# Autodesk Inventor assembly: Assembly1
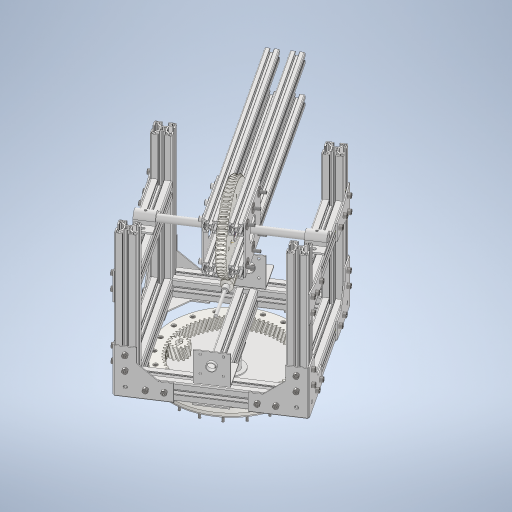
[picture p0: Inventor's stored thumbnail of the model, 512x512]
Saved by Autodesk Inventor 2024 (Build 280153000, 153)
## iProperties
Created: 2025-12-08
Part Number: Assembly1
Document SubType Name: Assembly
Designer: schar
Author: schar
## Documents named in this file (30)
- C:\Users\schar\Desktop\projectBlueprint\AMSTS\hardware\Assembly1.iam
- C:\Users\schar\Desktop\projectBlueprint\AMSTS\hardware\3030_200.ipt
- C:\Users\schar\Desktop\projectBlueprint\AMSTS\hardware\Connect2x3030_m6.ipt
- C:\Users\schar\Desktop\projectBlueprint\AMSTS\hardware\3030_tnut_m6.ipt
- C:\Users\schar\Documents\Inventor\Content Center Files\R2024\en-US\AS 1420\AS 1420 - 1973 - M5 x 10.ipt
- C:\Users\schar\Desktop\projectBlueprint\AMSTS\hardware\3030_260.ipt
- C:\Users\schar\Desktop\projectBlueprint\AMSTS\hardware\3030_connector_assembled.iam
- C:\Users\schar\Desktop\projectBlueprint\AMSTS\hardware\3030_connector_assembled_MIR.iam
- C:\Users\schar\Desktop\projectBlueprint\AMSTS\hardware\3030_connector_assembled_MIR1.iam
- C:\Users\schar\Desktop\projectBlueprint\AMSTS\hardware\3030_connector_assembled_MIR_MIR.iam
- C:\Users\schar\Desktop\projectBlueprint\AMSTS\hardware\3030_T_connector_assembled.iam
- C:\Users\schar\Desktop\projectBlueprint\AMSTS\hardware\3030_T_connector_assembled_MIR1.iam
- C:\Users\schar\Desktop\projectBlueprint\AMSTS\hardware\NEMA 17 - MS17HD2.iam
- C:\Users\schar\Desktop\projectBlueprint\AMSTS\hardware\wormgear_pol_base.iam
- C:\Users\schar\Desktop\projectBlueprint\AMSTS\hardware\base_axis_static_12mm.ipt
- C:\Users\schar\Desktop\projectBlueprint\AMSTS\hardware\base_axis_12mm.ipt
- C:\Users\schar\Desktop\projectBlueprint\AMSTS\hardware\NEMA17-3030-m6-holder.ipt
- C:\Users\schar\Desktop\projectBlueprint\AMSTS\hardware\3030_tnut_m6_main.ipt
- C:\Users\schar\Desktop\projectBlueprint\AMSTS\hardware\basis-bearing-3030-m6-holder.ipt
- C:\Users\schar\Desktop\projectBlueprint\AMSTS\hardware\wormgear_axis_6mm.ipt
- C:\Users\schar\Desktop\projectBlueprint\AMSTS\hardware\wormgear_worm_axes_holder.ipt
- C:\Users\schar\Desktop\projectBlueprint\AMSTS\hardware\bearing_shaft_base_mount.ipt
- C:\Users\schar\Desktop\projectBlueprint\AMSTS\hardware\az_rot_plate.iam
- C:\Users\schar\Desktop\projectBlueprint\AMSTS\hardware\transversal-2l-stabilizer.ipt
- C:\Users\schar\Desktop\projectBlueprint\AMSTS\hardware\the_part_that_holds_everything_together.ipt
- C:\Users\schar\Desktop\projectBlueprint\AMSTS\hardware\6901.iam
- C:\Users\schar\Desktop\projectBlueprint\AMSTS\hardware\2020_400.ipt
- C:\Users\schar\Desktop\projectBlueprint\AMSTS\hardware\mount_plate_4x2020.ipt
- C:\Users\schar\Documents\Inventor\Content Center Files\R2024\en-US\DIN 9021\DIN 9021 - 5,3.ipt
- C:\Users\schar\Desktop\projectBlueprint\AMSTS\hardware\m5x70.ipt
## Components (105 placed, 29 different names)
1. wormgear_axis_6mm:1 — Mate:61, Mate:62, Mate:63, Mate:64, Mate:65
2. wormgear_worm_axes_holder:1 — Mate:64, Mate:65, Rotational:26
3. 3030_tnut_m6_main:17 — Rotational:21
4. 3030_tnut_m6_main:18 — Rotational:22
5. bearing_shaft_base_mount:1 — Mate:102, Flush:37, Flush:38, Rotational:21, Rotational:22, Mate:103, Rotational:25
6. az_rot_plate:1 [sub-assembly] — Mate:103, Tangent:1, Rotational:23, Rotational:24
7. transversal-2l-stabilizer:1 — Mate:104, Mate:105, Mate:106
8. the_part_that_holds_everything_together:1 — Rotational:24, Rotational:25
9. 6901:1 [sub-assembly] — Rotational:23
10. 2020_400:1 — Mate:109, Mate:113, Mate:114, Mate:121
11. 2020_400:2 — Mate:107, Mate:117, Mate:118, Mate:122, Mate:123
12. 2020_400:3 — Mate:110, Mate:111, Mate:112, Mate:124
13. 2020_400:4 — Mate:108, Mate:115, Mate:116, Mate:119, Mate:120
14. mount_plate_4x2020:1 — Mate:119, Mate:120, Mate:121, Mate:125, Mate:127
15. mount_plate_4x2020:2 — Mate:122, Mate:123, Mate:124, Mate:130
16. 3030_200:1 — Mate:1, Mate:2, Flush:1, Flush:2, Mate:4, Flush:5, Flush:6, Symmetry:1, Mate:30, Mate:45, Flush:18, Mate:48
17. 3030_200:2 — Mate:3, Flush:3, Flush:4, Mate:6, Flush:9, Flush:10, Symmetry:2
18. Connect2x3030_m6:1 — Mate:1, Mate:2, Flush:1, Flush:2, Mate:3, Flush:3, Flush:4, Rigid:1, Rotational:5, Rotational:6, Rotational:7, Insert:11, Insert:12, Insert:14, Insert:15, Mate:19, Mate:20, Mate:21, Mate:36, Mate:37
19. Connect2x3030_m6:2 — Mate:4, Flush:5, Flush:6, Mate:5, Flush:7, Flush:8, Rotational:1, Rotational:2, Rotational:3, Rotational:4, Insert:6, Insert:7, Insert:9, Insert:10, Mate:10, Mate:11, Mate:12, Mate:32, Mate:33
20. Connect2x3030_m6:3 — Mate:8, Flush:11, Flush:12, Rotational:12, Rotational:13, Rotational:14, Rotational:15, Insert:1, Insert:2, Insert:4, Insert:5, Mate:13, Mate:14, Mate:15, Mate:40, Mate:41
21. Connect2x3030_m6:4 — Mate:6, Flush:9, Flush:10, Mate:7, Flush:13, Mate:9, Flush:14, Rotational:8, Rotational:9, Rotational:10, Rotational:11, Insert:16, Insert:17, Insert:18, Insert:20, Mate:16, Mate:17, Mate:18, Mate:23, Flush:15, Mate:25
22. 3030_200:3 — Mate:5, Flush:7, Flush:8, Mate:8, Flush:11, Flush:12, Symmetry:2, Mate:52, Angle:1, Mate:104, Mate:106
23. 3030_200:4 — Flush:13, Mate:9, Flush:14, Symmetry:1, Mate:53, Flush:23
24. 3030_connector_assembled:1 [sub-assembly] — Mate:24, Mate:25, Mate:26
25. 3030_connector_assembled:2 [sub-assembly] — Mate:22, Mate:23, Flush:15, Mate:26
26. 3030_connector_assembled_MIR:1 [sub-assembly] — Mate:27, Mate:39, Mate:40
27. 3030_connector_assembled_MIR:2 [sub-assembly] — Mate:27, Mate:38, Mate:41
28. 3030_connector_assembled_MIR1:1 [sub-assembly] — Mate:28, Mate:34, Mate:37
29. 3030_connector_assembled_MIR1:2 [sub-assembly] — Mate:28, Mate:35, Mate:36
30. 3030_connector_assembled_MIR_MIR:1 [sub-assembly] — Mate:29, Mate:30, Mate:33
31. 3030_connector_assembled_MIR_MIR:2 [sub-assembly] — Mate:29, Mate:31, Mate:32, Mate:105
32. 3030_260:1 — Mate:10, Mate:11, Mate:12, Mate:31, Mate:49, Flush:20
33. 3030_260:2 — Mate:13, Mate:14, Mate:15, Mate:38, Mate:39, Mate:42, Flush:16
34. 3030_260:3 — Mate:16, Mate:17, Mate:18, Mate:22, Mate:24, Mate:43, Flush:17
35. 3030_260:4 — Mate:19, Mate:20, Mate:21, Mate:34, Mate:35, Mate:50, Flush:21
36. NEMA 17 - MS17HD2:1 [sub-assembly] — Rotational:19, Rotational:20, Mate:61, Mate:62
37. wormgear_pol_base:1 [sub-assembly] — Rigid:2, Mate:63, Rotational:26, Mate:107, Mate:108, Mate:109, Mate:110, Mate:111, Mate:112, Mate:113, Mate:114, Mate:115, Mate:116, Mate:117, Mate:118
38. base_axis_static_12mm:1 — Flush:30, Mate:57, Insert:22
39. base_axis_static_12mm:2 — Mate:58, Flush:31, Flush:32, Insert:21
40. base_axis_12mm:1 — Insert:21, Insert:22, Rigid:2
41. basis-bearing-3030-m6-holder:1 — Mate:60, Flush:36, Insert:23, Insert:24
42. NEMA17-3030-m6-holder:1 — Mate:59, Flush:33, Insert:25, Insert:26, Rotational:19, Rotational:20
43. 3030_T_connector_assembled:1 [sub-assembly] — Mate:43, Flush:17, Mate:56, Flush:29
44. 3030_T_connector_assembled:2 [sub-assembly] — Mate:42, Flush:16, Flush:26
45. 3030_T_connector_assembled_MIR1:1 [sub-assembly] — Mate:50, Flush:21, Mate:55, Flush:27, Flush:28
46. 3030_T_connector_assembled_MIR1:2 [sub-assembly] — Mate:49, Flush:20, Mate:54, Flush:24, Flush:25
47. 3030_T_connector_assembled:3 [sub-assembly] — Mate:45, Flush:18, Mate:47, Flush:19
48. 3030_200:5 — Mate:47, Mate:48, Flush:19, Mate:52, Flush:22, Mate:59, Flush:33, Mate:60, Flush:36, Mate:102, Flush:37, Flush:38
49. 3030_T_connector_assembled:4 [sub-assembly] — Mate:53, Flush:22, Flush:23
50. 3030_200:6 — Mate:55, Flush:27, Flush:28, Mate:56, Flush:29, Flush:30, Mate:57
51. 3030_200:7 — Mate:54, Flush:24, Flush:25, Flush:26, Mate:58, Flush:31, Flush:32
52. 3030_tnut_m6:1 — Rotational:12
53. 3030_tnut_m6:2 — Rotational:11
54. 3030_tnut_m6:3 — Rigid:1
55. 3030_tnut_m6:4 — Rotational:1
56. 3030_tnut_m6:5 — Rotational:13
57. 3030_tnut_m6:6 — Rotational:10
58. 3030_tnut_m6:7 — Rotational:5
59. 3030_tnut_m6:8 — Rotational:2
60. 3030_tnut_m6:9 — Rotational:15
61. 3030_tnut_m6:10 — Rotational:8
62. 3030_tnut_m6:11 — Rotational:6
63. 3030_tnut_m6:12 — Rotational:4
64. 3030_tnut_m6:13 — Rotational:14
65. 3030_tnut_m6:14 — Rotational:9
66. 3030_tnut_m6:15 — Rotational:7
67. 3030_tnut_m6:16 — Rotational:3
68. AS 1420 - Metric M5 x 10:1 — Insert:1
69. AS 1420 - Metric M5 x 10:2 — Insert:2
70. AS 1420 - Metric M5 x 10:4 — Insert:4
71. AS 1420 - Metric M5 x 10:5 — Insert:5
72. AS 1420 - Metric M5 x 10:6 — Insert:6
73. AS 1420 - Metric M5 x 10:7 — Insert:7
74. AS 1420 - Metric M5 x 10:9 — Insert:9
75. AS 1420 - Metric M5 x 10:10 — Insert:10
76. AS 1420 - Metric M5 x 10:11 — Insert:11
77. AS 1420 - Metric M5 x 10:12 — Insert:12
78. AS 1420 - Metric M5 x 10:14 — Insert:14
79. AS 1420 - Metric M5 x 10:15 — Insert:15
80. AS 1420 - Metric M5 x 10:16 — Insert:16
81. AS 1420 - Metric M5 x 10:17 — Insert:17
82. AS 1420 - Metric M5 x 10:18 — Insert:18
83. AS 1420 - Metric M5 x 10:20 — Insert:20
84. AS 1420 - Metric M5 x 10:21 — Insert:23
85. AS 1420 - Metric M5 x 10:22 — Insert:24
86. AS 1420 - Metric M5 x 10:23 — Insert:25
87. AS 1420 - Metric M5 x 10:24 — Insert:26
88. DIN 9021 5,3:9
89. DIN 9021 5,3:13
90. DIN 9021 5,3:14
91. DIN 9021 5,3:15
92. DIN 9021 5,3:16
93. DIN 9021 5,3:17 — Mate:129, Mate:130
94. DIN 9021 5,3:1
95. DIN 9021 5,3:18
96. DIN 9021 5,3:19
97. DIN 9021 5,3:20
98. DIN 9021 5,3:21 — Mate:126, Mate:127, Mate:128
99. DIN 9021 5,3:22
100. m5x70:1 — Mate:125, Mate:126, Mate:128, Mate:129
101. m5x70:2
102. m5x70:3
103. m5x70:4
104. m5x70:5
105. m5x70:6
## Component patterns: (6 elements, first: DIN 9021 5,3:9), (6 elements, first: DIN 9021 5,3:1), (6 elements, first: m5x70:1)
## Relationships (178: Mate 91, Flush 36, RevoluteJoint 23, Insert 22, WeldJoint 2, Symmetry 2, Angle 1, Tangent 1)
- Mate:1: 3030_200:1 ↔ Connect2x3030_m6:1
- Mate:2: 3030_200:1 ↔ Connect2x3030_m6:1
- Flush:1: 3030_200:1 ↔ Connect2x3030_m6:1
- Flush:2 (30 mm): 3030_200:1 ↔ Connect2x3030_m6:1
- Mate:3: 3030_200:2 ↔ Connect2x3030_m6:1
- Flush:3 (30 mm): 3030_200:2 ↔ Connect2x3030_m6:1
- Flush:4: 3030_200:2 ↔ Connect2x3030_m6:1
- Mate:4: 3030_200:1 ↔ Connect2x3030_m6:2
- Flush:5 (-30 mm): 3030_200:1 ↔ Connect2x3030_m6:2
- Flush:6: 3030_200:1 ↔ Connect2x3030_m6:2
- Mate:5: Connect2x3030_m6:2 ↔ 3030_200:3
- Flush:7 (30 mm): Connect2x3030_m6:2 ↔ 3030_200:3
- Flush:8: Connect2x3030_m6:2 ↔ 3030_200:3
- Mate:6: 3030_200:2 ↔ Connect2x3030_m6:4
- Flush:9 (-30 mm): 3030_200:2 ↔ Connect2x3030_m6:4
- Flush:10: 3030_200:2 ↔ Connect2x3030_m6:4
- Mate:7: Connect2x3030_m6:4
- Mate:8: Connect2x3030_m6:3 ↔ 3030_200:3
- Flush:11 (-30 mm): Connect2x3030_m6:3 ↔ 3030_200:3
- Flush:12: Connect2x3030_m6:3 ↔ 3030_200:3
- Flush:13: Connect2x3030_m6:4 ↔ 3030_200:4
- Mate:9: Connect2x3030_m6:4 ↔ 3030_200:4
- Flush:14 (-30 mm): Connect2x3030_m6:4 ↔ 3030_200:4
- Rotational:1 [RevoluteJoint] (-0.357 mm): Connect2x3030_m6:2 ↔ 3030_tnut_m6:4
- Rotational:2 [RevoluteJoint] (-0.357 mm): Connect2x3030_m6:2 ↔ 3030_tnut_m6:8
- Rotational:3 [RevoluteJoint] (-0.357 mm): Connect2x3030_m6:2 ↔ 3030_tnut_m6:16
- Rotational:4 [RevoluteJoint] (-0.357 mm): Connect2x3030_m6:2 ↔ 3030_tnut_m6:12
- Rigid:1 [WeldJoint] (-0.357 mm): Connect2x3030_m6:1 ↔ 3030_tnut_m6:3
- Rotational:5 [RevoluteJoint] (-0.357 mm): Connect2x3030_m6:1 ↔ 3030_tnut_m6:7
- Rotational:6 [RevoluteJoint] (-0.357 mm): Connect2x3030_m6:1 ↔ 3030_tnut_m6:11
- Rotational:7 [RevoluteJoint] (-0.357 mm): Connect2x3030_m6:1 ↔ 3030_tnut_m6:15
- Rotational:8 [RevoluteJoint] (-0.357 mm): Connect2x3030_m6:4 ↔ 3030_tnut_m6:10
- Rotational:9 [RevoluteJoint] (-0.357 mm): Connect2x3030_m6:4 ↔ 3030_tnut_m6:14
- Rotational:10 [RevoluteJoint] (-0.357 mm): Connect2x3030_m6:4 ↔ 3030_tnut_m6:6
- Rotational:11 [RevoluteJoint] (-0.357 mm): Connect2x3030_m6:4 ↔ 3030_tnut_m6:2
- Rotational:12 [RevoluteJoint] (-0.357 mm): Connect2x3030_m6:3 ↔ 3030_tnut_m6:1
- Rotational:13 [RevoluteJoint]: Connect2x3030_m6:3 ↔ 3030_tnut_m6:5
- Rotational:14 [RevoluteJoint] (-0.357 mm): Connect2x3030_m6:3 ↔ 3030_tnut_m6:13
- Rotational:15 [RevoluteJoint] (-0.357 mm): Connect2x3030_m6:3 ↔ 3030_tnut_m6:9
- Insert:1: Connect2x3030_m6:3 ↔ AS 1420 - Metric M5 x 10:1
- Insert:2: Connect2x3030_m6:3 ↔ AS 1420 - Metric M5 x 10:2
- Insert:4: Connect2x3030_m6:3 ↔ AS 1420 - Metric M5 x 10:4
- Insert:5: Connect2x3030_m6:3 ↔ AS 1420 - Metric M5 x 10:5
- Insert:6: Connect2x3030_m6:2 ↔ AS 1420 - Metric M5 x 10:6
- Insert:7: Connect2x3030_m6:2 ↔ AS 1420 - Metric M5 x 10:7
- Insert:9: Connect2x3030_m6:2 ↔ AS 1420 - Metric M5 x 10:9
- Insert:10: Connect2x3030_m6:2 ↔ AS 1420 - Metric M5 x 10:10
- Insert:11: Connect2x3030_m6:1 ↔ AS 1420 - Metric M5 x 10:11
- Insert:12: Connect2x3030_m6:1 ↔ AS 1420 - Metric M5 x 10:12
- Insert:14: Connect2x3030_m6:1 ↔ AS 1420 - Metric M5 x 10:14
- Insert:15: Connect2x3030_m6:1 ↔ AS 1420 - Metric M5 x 10:15
- Insert:16: Connect2x3030_m6:4 ↔ AS 1420 - Metric M5 x 10:16
- Insert:17: Connect2x3030_m6:4 ↔ AS 1420 - Metric M5 x 10:17
- Insert:18: Connect2x3030_m6:4 ↔ AS 1420 - Metric M5 x 10:18
- Insert:20: Connect2x3030_m6:4 ↔ AS 1420 - Metric M5 x 10:20
- Mate:10: Connect2x3030_m6:2 ↔ 3030_260:1
- Mate:11: Connect2x3030_m6:2 ↔ 3030_260:1
- Mate:12: Connect2x3030_m6:2 ↔ 3030_260:1
- Mate:13: Connect2x3030_m6:3 ↔ 3030_260:2
- Mate:14: Connect2x3030_m6:3 ↔ 3030_260:2
- Mate:15: Connect2x3030_m6:3 ↔ 3030_260:2
- Mate:16: Connect2x3030_m6:4 ↔ 3030_260:3
- Mate:17: Connect2x3030_m6:4 ↔ 3030_260:3
- Mate:18: Connect2x3030_m6:4 ↔ 3030_260:3
- Mate:19: Connect2x3030_m6:1 ↔ 3030_260:4
- Mate:20: Connect2x3030_m6:1 ↔ 3030_260:4
- Mate:21: Connect2x3030_m6:1 ↔ 3030_260:4
- Symmetry:1: 3030_200:1 ↔ 3030_200:4
- Mate:22: 3030_connector_assembled:2 ↔ 3030_260:3
- Mate:23: Connect2x3030_m6:4 ↔ 3030_connector_assembled:2
- Flush:15: Connect2x3030_m6:4 ↔ 3030_connector_assembled:2
- Mate:24: 3030_connector_assembled:1 ↔ 3030_260:3
- Mate:25: Connect2x3030_m6:4 ↔ 3030_connector_assembled:1
- Mate:26: 3030_connector_assembled:1 ↔ 3030_connector_assembled:2
- Symmetry:2: 3030_200:2 ↔ 3030_200:3
- Mate:27: 3030_connector_assembled_MIR:1 ↔ 3030_connector_assembled_MIR:2
- Mate:28: 3030_connector_assembled_MIR1:1 ↔ 3030_connector_assembled_MIR1:2
- Mate:29: 3030_connector_assembled_MIR_MIR:1 ↔ 3030_connector_assembled_MIR_MIR:2
- Mate:30: 3030_200:1 ↔ 3030_connector_assembled_MIR_MIR:1
- Mate:31: 3030_connector_assembled_MIR_MIR:2 ↔ 3030_260:1
- Mate:32: Connect2x3030_m6:2 ↔ 3030_connector_assembled_MIR_MIR:2
- Mate:33: Connect2x3030_m6:2 ↔ 3030_connector_assembled_MIR_MIR:1
- Mate:34: 3030_connector_assembled_MIR1:1 ↔ 3030_260:4
- Mate:35: 3030_connector_assembled_MIR1:2 ↔ 3030_260:4
- Mate:36: Connect2x3030_m6:1 ↔ 3030_connector_assembled_MIR1:2
- Mate:37: Connect2x3030_m6:1 ↔ 3030_connector_assembled_MIR1:1
- Mate:38: 3030_connector_assembled_MIR:2 ↔ 3030_260:2
- Mate:39: 3030_connector_assembled_MIR:1 ↔ 3030_260:2
- Mate:40: Connect2x3030_m6:3 ↔ 3030_connector_assembled_MIR:1
- Mate:41: Connect2x3030_m6:3 ↔ 3030_connector_assembled_MIR:2
- Mate:42: 3030_260:2 ↔ 3030_T_connector_assembled:2
- Flush:16: 3030_260:2 ↔ 3030_T_connector_assembled:2
- Mate:43: 3030_260:3 ↔ 3030_T_connector_assembled:1
- Flush:17: 3030_260:3 ↔ 3030_T_connector_assembled:1
- Mate:45: 3030_200:1 ↔ 3030_T_connector_assembled:3
- Flush:18: 3030_200:1 ↔ 3030_T_connector_assembled:3
- Mate:47: 3030_T_connector_assembled:3 ↔ 3030_200:5
- Mate:48: 3030_200:1 ↔ 3030_200:5
- Flush:19: 3030_T_connector_assembled:3 ↔ 3030_200:5
- Mate:49: 3030_260:1 ↔ 3030_T_connector_assembled_MIR1:2
- Flush:20: 3030_260:1 ↔ 3030_T_connector_assembled_MIR1:2
- Mate:50: 3030_260:4 ↔ 3030_T_connector_assembled_MIR1:1
- Flush:21: 3030_260:4 ↔ 3030_T_connector_assembled_MIR1:1
- Mate:52 (85 mm): 3030_200:3 ↔ 3030_200:5
- Mate:53: 3030_200:4 ↔ 3030_T_connector_assembled:4
- Flush:22: 3030_200:5 ↔ 3030_T_connector_assembled:4
- Flush:23: 3030_200:4 ↔ 3030_T_connector_assembled:4
- Mate:54: 3030_T_connector_assembled_MIR1:2 ↔ 3030_200:7
- Flush:24: 3030_T_connector_assembled_MIR1:2 ↔ 3030_200:7
- Flush:25 (-30 mm): 3030_T_connector_assembled_MIR1:2 ↔ 3030_200:7
- Flush:26: 3030_T_connector_assembled:2 ↔ 3030_200:7
- Mate:55: 3030_T_connector_assembled_MIR1:1 ↔ 3030_200:6
- Flush:27: 3030_T_connector_assembled_MIR1:1 ↔ 3030_200:6
- Flush:28 (30 mm): 3030_T_connector_assembled_MIR1:1 ↔ 3030_200:6
- Mate:56: 3030_T_connector_assembled:1 ↔ 3030_200:6
- Flush:29: 3030_T_connector_assembled:1 ↔ 3030_200:6
- Flush:30: base_axis_static_12mm:1 ↔ 3030_200:6
- Mate:57: base_axis_static_12mm:1 ↔ 3030_200:6
- Mate:58: base_axis_static_12mm:2 ↔ 3030_200:7
- Flush:31: base_axis_static_12mm:2 ↔ 3030_200:7
- Flush:32 (-75 mm): base_axis_static_12mm:2 ↔ 3030_200:7
- Insert:21: base_axis_static_12mm:2 ↔ base_axis_12mm:1
- Insert:22: base_axis_static_12mm:1 ↔ base_axis_12mm:1
- Rigid:2 [WeldJoint] (5 mm): wormgear_pol_base:1 ↔ base_axis_12mm:1
- Mate:59: NEMA17-3030-m6-holder:1 ↔ 3030_200:5
- Flush:33 (-10 mm): NEMA17-3030-m6-holder:1 ↔ 3030_200:5
- Mate:60: basis-bearing-3030-m6-holder:1 ↔ 3030_200:5
- Flush:36 (-10 mm): basis-bearing-3030-m6-holder:1 ↔ 3030_200:5
- Insert:23: basis-bearing-3030-m6-holder:1 ↔ AS 1420 - Metric M5 x 10:21
- Insert:24: basis-bearing-3030-m6-holder:1 ↔ AS 1420 - Metric M5 x 10:22
- Insert:25: NEMA17-3030-m6-holder:1 ↔ AS 1420 - Metric M5 x 10:23
- Insert:26: NEMA17-3030-m6-holder:1 ↔ AS 1420 - Metric M5 x 10:24
- Rotational:19 [RevoluteJoint]: NEMA 17 - MS17HD2:1 ↔ NEMA17-3030-m6-holder:1
- Rotational:20 [RevoluteJoint]: NEMA 17 - MS17HD2:1 ↔ NEMA17-3030-m6-holder:1
- Mate:61: wormgear_axis_6mm:1 ↔ NEMA 17 - MS17HD2:1
- Mate:62: wormgear_axis_6mm:1 ↔ NEMA 17 - MS17HD2:1
- Mate:63: wormgear_axis_6mm:1 ↔ wormgear_pol_base:1
- Mate:64: wormgear_axis_6mm:1 ↔ wormgear_worm_axes_holder:1
- Mate:65: wormgear_axis_6mm:1 ↔ wormgear_worm_axes_holder:1
- Mate:102: bearing_shaft_base_mount:1 ↔ 3030_200:5
- Flush:37 (79 mm): bearing_shaft_base_mount:1 ↔ 3030_200:5
- Flush:38: bearing_shaft_base_mount:1 ↔ 3030_200:5
- Rotational:21 [RevoluteJoint] (0.357 mm): 3030_tnut_m6_main:17 ↔ bearing_shaft_base_mount:1
- Rotational:22 [RevoluteJoint] (0.357 mm): 3030_tnut_m6_main:18 ↔ bearing_shaft_base_mount:1
- Mate:103: bearing_shaft_base_mount:1 ↔ az_rot_plate:1
- Angle:1 (0 deg): 3030_200:3
- Tangent:1: az_rot_plate:1
- Mate:104: transversal-2l-stabilizer:1 ↔ 3030_200:3
- Mate:105 (35 mm): transversal-2l-stabilizer:1 ↔ 3030_connector_assembled_MIR_MIR:2
- Mate:106: transversal-2l-stabilizer:1 ↔ 3030_200:3
- Rotational:23 [RevoluteJoint]: az_rot_plate:1 ↔ 6901:1
- Rotational:24 [RevoluteJoint]: az_rot_plate:1 ↔ the_part_that_holds_everything_together:1
- Rotational:25 [RevoluteJoint]: bearing_shaft_base_mount:1 ↔ the_part_that_holds_everything_together:1
- Rotational:26 [RevoluteJoint]: wormgear_worm_axes_holder:1 ↔ wormgear_pol_base:1
- Mate:107: 2020_400:2 ↔ wormgear_pol_base:1
- Mate:108: 2020_400:4 ↔ wormgear_pol_base:1
- Mate:109: 2020_400:1 ↔ wormgear_pol_base:1
- Mate:110: 2020_400:3 ↔ wormgear_pol_base:1
- Mate:111: 2020_400:3 ↔ wormgear_pol_base:1
- Mate:112: 2020_400:3 ↔ wormgear_pol_base:1
- Mate:113: 2020_400:1 ↔ wormgear_pol_base:1
- Mate:114: 2020_400:1 ↔ wormgear_pol_base:1
- Mate:115: 2020_400:4 ↔ wormgear_pol_base:1
- Mate:116: 2020_400:4 ↔ wormgear_pol_base:1
- Mate:117: 2020_400:2 ↔ wormgear_pol_base:1
- Mate:118: 2020_400:2 ↔ wormgear_pol_base:1
- Mate:119: 2020_400:4 ↔ mount_plate_4x2020:1
- Mate:120: 2020_400:4 ↔ mount_plate_4x2020:1
- Mate:121: 2020_400:1 ↔ mount_plate_4x2020:1
- Mate:122: 2020_400:2 ↔ mount_plate_4x2020:2
- Mate:123: 2020_400:2 ↔ mount_plate_4x2020:2
- Mate:124: 2020_400:3 ↔ mount_plate_4x2020:2
- Mate:125: mount_plate_4x2020:1 ↔ m5x70:1
- Mate:126: DIN 9021 5,3:21 ↔ m5x70:1
- Mate:127: mount_plate_4x2020:1 ↔ DIN 9021 5,3:21
- Mate:128: DIN 9021 5,3:21 ↔ m5x70:1
- Mate:129: DIN 9021 5,3:17 ↔ m5x70:1
- Mate:130: mount_plate_4x2020:2 ↔ DIN 9021 5,3:17
